# Autodesk Inventor assembly: Arm 2.0 Assembly
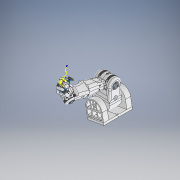
[picture p0: Inventor's stored thumbnail of the model, 180x180]
Saved by Autodesk Inventor 2017 SP1 (Build 210196100, 196)
## iProperties
Created: 2017-09-28
Part Number: Arm 2.0 Assembly
Document SubType Name: Assembly
Designer: Zach
Author: Zach
## Documents named in this file (39)
- C:\Users\Zach\Documents\GitHub\tr1\src\Body\Arm 2.0 Assembly\Arm 2.0 Assembly.iam
- C:\Users\Zach\Documents\GitHub\tr1\src\Body\Arm 2.0 Assembly\AA001.ipt
- C:\Users\Zach\Documents\GitHub\tr1\src\Body\Arm 2.0 Assembly\Steel Rod 8mm x 135mm.ipt
- C:\Users\Zach\Documents\GitHub\tr1\lib\22x8x8mm Bearing.ipt
- C:\Users\Zach\Documents\GitHub\tr1\src\Body\Arm 2.0 Assembly\AA002.ipt
- C:\Users\Zach\Documents\GitHub\tr1\src\Body\Arm 2.0 Assembly\AA003.ipt
- C:\Users\Zach\Documents\GitHub\tr1\src\Body\Arm 2.0 Assembly\AA004.ipt
- C:\Users\Zach\Documents\GitHub\tr1\src\Body\Arm 2.0 Assembly\AA005.ipt
- C:\Users\Zach\Documents\GitHub\tr1\src\Body\Arm 2.0 Assembly\AA006.ipt
- C:\Users\Zach\Documents\GitHub\tr1\src\Body\Arm 2.0 Assembly\AA007.ipt
- C:\Users\Zach\Documents\GitHub\tr1\lib\QS12MM250\QS12MM250.ipt
- C:\Users\Zach\Documents\GitHub\tr1\src\Body\Arm 2.0 Assembly\AA008.ipt
- C:\Users\Zach\Documents\GitHub\tr1\src\Body\Arm 2.0 Assembly\AA009.ipt
- C:\Users\Zach\Documents\GitHub\tr1\lib\13x4x5mm Bearing.ipt
- C:\Users\Zach\Documents\GitHub\tr1\src\Body\Arm 2.0 Assembly\AA010.ipt
- C:\Users\Zach\Documents\GitHub\tr1\src\Body\Arm 2.0 Assembly\AA011.ipt
- C:\Users\Zach\Documents\GitHub\tr1\src\Body\Arm 2.0 Assembly\AA012.ipt
- C:\Users\Zach\Documents\GitHub\tr1\src\Body\Arm 2.0 Assembly\Steel Rod 8mm x 100mm.ipt
- C:\Users\Zach\Documents\GitHub\tr1\src\Body\Arm 2.0 Assembly\AA013.ipt
- C:\Users\Zach\Documents\GitHub\tr1\src\Body\Arm 2.0 Assembly\AA014.ipt
- C:\Users\Zach\Documents\GitHub\tr1\src\Body\Arm 2.0 Assembly\AA015.ipt
- C:\Users\Zach\Documents\GitHub\tr1\src\Body\Arm 2.0 Assembly\AA016.ipt
- C:\Users\Zach\Documents\GitHub\tr1\src\Body\Arm 2.0 Assembly\AA017.ipt
- C:\Users\Zach\Documents\Inventor\Content Center Files\R2017\en-US\ISO 4762(2)\ISO 4762 - M4 x 20ISO.ipt
- C:\Users\Zach\Documents\Inventor\Content Center Files\R2017\en-US\ISO 4035(2)\ISO 4035 - M4 - ISO.ipt
- C:\Users\Zach\Documents\GitHub\tr1\lib\12V DC Motor 378-1.ipt
- C:\Users\Zach\Documents\GitHub\tr1\src\Body\Arm 2.0 Assembly\AA018.ipt
- C:\Users\Zach\Documents\Inventor\Content Center Files\R2017\en-US\ISO 4016\ISO 4016 - M5 x 25.ipt
- C:\Users\Zach\Documents\Inventor\Content Center Files\R2017\en-US\ISO 4017(1)\ISO 4017 - M5 x 12 - ISO.ipt
- C:\Users\Zach\Documents\Inventor\Content Center Files\R2017\en-US\ISO 4017(1)\ISO 4017 - M5 x 20 - ISO.ipt
- C:\Users\Zach\Documents\GitHub\tr1\src\Body\Arm 2.0 Assembly\AA019.ipt
- C:\Users\Zach\Documents\GitHub\tr1\src\Body\Arm 2.0 Assembly\AA020.ipt
- C:\Users\Zach\Documents\GitHub\tr1\src\Body\Arm 2.0 Assembly\AA021.ipt
- C:\Users\Zach\Documents\GitHub\tr1\src\Body\Arm 2.0 Assembly\AA022.ipt
- C:\Users\Zach\Documents\GitHub\tr1\src\Body\Arm 2.0 Assembly\Steel Rod 8mm x 80mm.ipt
- C:\Users\Zach\Documents\GitHub\tr1\src\Body\Arm 2.0 Assembly\AA023.ipt
- C:\Users\Zach\Documents\GitHub\BCN3D-Moveo\Autodesk Inventor files\Gripper B Assembly.iam
- C:\Users\Zach\Documents\GitHub\tr1\src\Body\Arm 2.0 Assembly\AA024.ipt
- C:\Users\Zach\Documents\GitHub\tr1\lib\Gearbox 8;1\Gearbox 8;1.iam
## Components (88 placed, 38 different names)
1. AA001:1 — Mate:1, Mate:3, Flush:1, Flush:2, Mate:7, Mate:9, Mate:10, Mate:11, Mate:58, Mate:59, Mate:60, Mate:61, Mate:62, Mate:63, Mate:82, Mate:83, Mate:84, Mate:101, Mate:102, Mate:104, Mate:105, Mate:138, Mate:139, Mate:140, Mate:141
2. AA002:2 — Flush:4, Mate:5, Mate:8, Mate:14, Mate:28, Mate:29, Mate:34
3. AA003:1 — Flush:4, Mate:5, Mate:6, Mate:7, Mate:8, Mate:27, Mate:32
4. AA004:1 — Mate:9, Mate:10, Mate:11, Mate:12, Mate:13, Mate:15, Mate:23, Mate:26
5. AA005:1 — Mate:26, Mate:99, Mate:100, Mate:103
6. AA006:1 — Mate:24, Mate:25, Mate:96, Mate:97, Mate:98
7. AA007:1 — Mate:19, Mate:20, Mate:99, Mate:100, Mate:103
8. AA007:2 — Mate:19, Mate:20, Mate:96, Mate:97, Mate:98
9. AA008:1 — Mate:27, Mate:28, Mate:29, Mate:30, Mate:31, Mate:33, Mate:35, Mate:36, Mate:39, Mate:41, Mate:43, Mate:46, Mate:47, Mate:131, Mate:132, Mate:135, Mate:137, Flush:11, Mate:167, Mate:213
10. AA008:2 — Mate:32, Mate:33, Mate:34, Mate:37, Mate:38, Mate:40, Mate:42, Mate:44, Mate:45, Mate:48, Mate:76, Mate:130, Mate:133, Mate:134, Mate:136, Flush:12, Mate:168, Mate:212, Mate:218, Mate:219, Mate:220
11. AA009:1 — Mate:30, Mate:31
12. AA010:1 — Mate:47, Mate:48, Mate:52, Mate:53, Mate:55, Flush:6, Mate:56, Flush:7, Flush:8, Mate:64, Mate:65, Mate:66, Mate:67, Mate:68, Mate:69, Mate:107, Mate:108, Mate:109, Mate:214
13. AA011:1 — Mate:49, Mate:50, Mate:51, Flush:9, Mate:79, Mate:81, Mate:113, Mate:114
14. AA012:1 — Mate:49, Mate:50, Mate:51, Mate:52, Mate:53, Flush:9, Mate:80, Mate:110, Mate:112, Mate:115
15. AA013:1 — Mate:58, Mate:59, Mate:60, Mate:148, Mate:149, Mate:150, Mate:151, Mate:152, Mate:153
16. AA013:2 — Mate:61, Mate:62, Mate:63, Mate:142, Mate:143, Mate:144, Mate:145, Mate:146, Mate:147
17. AA014:1 — Mate:64, Mate:65, Mate:66, Mate:160, Mate:161, Mate:162, Mate:163, Mate:164, Mate:165
18. AA014:2 — Mate:67, Mate:68, Mate:69, Mate:154, Mate:155, Mate:156, Mate:157, Mate:158, Mate:159
19. AA015:1 — Mate:166, Flush:11, Mate:167
20. AA015:2 — Mate:76, Flush:12, Mate:168
21. AA016:1 — Mate:79, Mate:80, Mate:81, Flush:10, Mate:111, Mate:112, Mate:113, Mate:116, Mate:124, Mate:125, Mate:127, Mate:129, Flush:14, Mate:170, Mate:215, Mate:216, Mate:217
22. AA016:2 — Flush:10, Mate:110, Mate:111, Mate:114, Mate:115, Mate:119, Mate:122, Mate:123, Mate:126, Mate:128, Flush:13, Mate:169, Mate:180, Mate:181
23. AA017:1 — Mate:82, Mate:83, Mate:84, Mate:85, Mate:86, Mate:91, Mate:92, Mate:95
24. AA018:1 — Mate:116, Flush:14, Mate:170
25. AA018:2 — Mate:119, Flush:13, Mate:169
26. AA019:1 — Mate:174, Mate:175, Mate:176, Mate:177, Mate:178, Mate:179, Mate:182, Mate:183, Mate:184, Mate:185, Flush:15, Flush:16, Flush:17, Mate:188, Mate:189, Mate:190, Mate:191, Mate:192, Mate:193
27. AA020:1 — Mate:171, Mate:172, Mate:173, Mate:175, Mate:194, Mate:196
28. AA021:1 — Mate:171, Mate:172, Mate:173, Mate:174, Mate:195
29. AA022:1 — Mate:176, Mate:177, Mate:181, Mate:200, Flush:18, Mate:203, Mate:204, Mate:206, Mate:209, Mate:210
30. AA022:2 — Mate:178, Mate:179, Mate:180, Flush:19, Mate:201, Mate:202, Mate:205, Mate:207, Mate:208, Mate:211
31. AA023:1 — Mate:188, Mate:189, Mate:193
32. AA023:2 — Mate:190, Mate:191, Mate:192
33. AA024:1 — Mate:200, Flush:18, Mate:203
34. AA024:2 — Flush:19, Mate:201, Mate:202
35. Gearbox 8;1:1 [sub-assembly] — Mate:212, Mate:213, Mate:214
36. Gripper B Assembly:1 [sub-assembly] — Mate:194, Mate:195, Mate:196
37. 13x4x5mm Bearing:1 — Mate:35, Mate:36
38. 13x4x5mm Bearing:2 — Mate:37, Mate:38
39. 13x4x5mm Bearing:3 — Mate:40, Mate:44
40. 13x4x5mm Bearing:4 — Mate:39, Mate:43
41. 13x4x5mm Bearing:5 — Mate:42, Mate:45
42. 13x4x5mm Bearing:6 — Mate:41, Mate:46
43. 13x4x5mm Bearing:7 — Mate:85, Mate:86, Mate:87, Mate:88, Mate:94
44. 13x4x5mm Bearing:8 — Mate:89, Mate:90
45. 13x4x5mm Bearing:9 — Mate:87, Mate:88, Mate:89, Mate:90
46. 22x8x8mm Bearing:1 — Mate:3, Flush:1, Flush:3
47. 22x8x8mm Bearing:2 — Flush:2, Mate:105
48. 22x8x8mm Bearing:3 — Mate:55, Flush:6, Mate:57
49. 22x8x8mm Bearing:4 — Mate:56, Flush:7
50. 22x8x8mm Bearing:5 — Mate:186, Flush:16
51. 22x8x8mm Bearing:6 — Mate:187, Flush:17
52. QS12MM250:1 — Mate:23, Mate:24, Mate:25
53. Steel Rod 8mm x 135mm:1 — Mate:1, Flush:3, Mate:6
54. Steel Rod 8mm x 100mm:1 — Mate:57, Flush:8
55. Steel Rod 8mm x 80mm:1 — Mate:185, Flush:15, Mate:186, Mate:187
56. 12V DC Motor 378-1:1 — Mate:101, Mate:102, Mate:104
57. 12V DC Motor 378-1:2 — Mate:107, Mate:108, Mate:109
58. 12V DC Motor 378-1:3 — Mate:182, Mate:183, Mate:184
59. 12V DC Motor 378-1:4 — Mate:215, Mate:216, Mate:217
60. 12V DC Motor 378-1:5 — Mate:218, Mate:219, Mate:220
61. ISO 4762 M4 x 20:1 — Mate:91, Mate:92, Mate:93
62. ISO 4035 M4:1 — Mate:93, Mate:94, Mate:95
63. ISO 4016 M5 x 25:1 — Mate:122, Mate:123
64. ISO 4016 M5 x 25:2 — Mate:124, Mate:125
65. ISO 4016 M5 x 25:3 — Mate:127, Mate:129
66. ISO 4016 M5 x 25:4 — Mate:126, Mate:128
67. ISO 4016 M5 x 25:5 — Mate:130, Mate:133
68. ISO 4016 M5 x 25:6 — Mate:131, Mate:132
69. ISO 4016 M5 x 25:7 — Mate:134, Mate:136
70. ISO 4016 M5 x 25:8 — Mate:135, Mate:137, Mate:166
71. ISO 4016 M5 x 25:9 — Mate:138, Mate:139
72. ISO 4016 M5 x 25:10 — Mate:140, Mate:141
73. ISO 4016 M5 x 25:11 — Mate:204, Mate:206
74. ISO 4016 M5 x 25:12 — Mate:205, Mate:207
75. ISO 4017 M5 x 20:1 — Mate:146, Mate:147
76. ISO 4017 M5 x 20:2 — Mate:144, Mate:145
77. ISO 4017 M5 x 20:3 — Mate:142, Mate:143
78. ISO 4017 M5 x 20:4 — Mate:148, Mate:149
79. ISO 4017 M5 x 20:5 — Mate:152, Mate:153
80. ISO 4017 M5 x 20:6 — Mate:150, Mate:151
81. ISO 4017 M5 x 12:1 — Mate:154, Mate:155
82. ISO 4017 M5 x 12:2 — Mate:156, Mate:158
83. ISO 4017 M5 x 12:3 — Mate:157, Mate:159
84. ISO 4017 M5 x 12:4 — Mate:160, Mate:161
85. ISO 4017 M5 x 12:5 — Mate:162, Mate:163
86. ISO 4017 M5 x 12:6 — Mate:164, Mate:165
87. ISO 4016 M5 x 25:13 — Mate:209, Mate:210
88. ISO 4016 M5 x 25:14 — Mate:208, Mate:211
## Relationships (214: Mate 196, Flush 18)
- Mate:1: AA001:1 ↔ Steel Rod 8mm x 135mm:1
- Mate:3: AA001:1 ↔ 22x8x8mm Bearing:1
- Flush:1: AA001:1 ↔ 22x8x8mm Bearing:1
- Flush:2: AA001:1 ↔ 22x8x8mm Bearing:2
- Flush:3 (-2.5 mm): 22x8x8mm Bearing:1 ↔ Steel Rod 8mm x 135mm:1
- Flush:4: AA002:2 ↔ AA003:1
- Mate:5: AA002:2 ↔ AA003:1
- Mate:6: AA003:1 ↔ Steel Rod 8mm x 135mm:1
- Mate:7 (0.75 mm): AA001:1 ↔ AA003:1
- Mate:8: AA002:2 ↔ AA003:1
- Mate:9: AA001:1 ↔ AA004:1
- Mate:10: AA001:1 ↔ AA004:1
- Mate:11: AA001:1 ↔ AA004:1
- Mate:12: AA004:1
- Mate:13: AA004:1
- Mate:14: AA002:2
- Mate:15: AA004:1
- Mate:19: AA007:1 ↔ AA007:2
- Mate:20: AA007:1 ↔ AA007:2
- Mate:23: AA004:1 ↔ QS12MM250:1
- Mate:24: AA006:1 ↔ QS12MM250:1
- Mate:25: AA006:1 ↔ QS12MM250:1
- Mate:26 (30 mm): AA004:1 ↔ AA005:1
- Mate:27: AA003:1 ↔ AA008:1
- Mate:28: AA002:2 ↔ AA008:1
- Mate:29: AA002:2 ↔ AA008:1
- Mate:30: AA008:1 ↔ AA009:1
- Mate:31: AA008:1 ↔ AA009:1
- Mate:32: AA003:1 ↔ AA008:2
- Mate:33: AA008:1 ↔ AA008:2
- Mate:34: AA002:2 ↔ AA008:2
- Mate:35: AA008:1 ↔ 13x4x5mm Bearing:1
- Mate:36: AA008:1 ↔ 13x4x5mm Bearing:1
- Mate:37: AA008:2 ↔ 13x4x5mm Bearing:2
- Mate:38: AA008:2 ↔ 13x4x5mm Bearing:2
- Mate:39: AA008:1 ↔ 13x4x5mm Bearing:4
- Mate:40: AA008:2 ↔ 13x4x5mm Bearing:3
- Mate:41: AA008:1 ↔ 13x4x5mm Bearing:6
- Mate:42: AA008:2 ↔ 13x4x5mm Bearing:5
- Mate:43: AA008:1 ↔ 13x4x5mm Bearing:4
- Mate:44: AA008:2 ↔ 13x4x5mm Bearing:3
- Mate:45: AA008:2 ↔ 13x4x5mm Bearing:5
- Mate:46: AA008:1 ↔ 13x4x5mm Bearing:6
- Mate:47: AA008:1 ↔ AA010:1
- Mate:48 (2.5 mm): AA008:2 ↔ AA010:1
- Mate:49: AA011:1 ↔ AA012:1
- Mate:50: AA011:1 ↔ AA012:1
- Mate:51: AA011:1 ↔ AA012:1
- Mate:52: AA010:1 ↔ AA012:1
- Mate:53 (1.75 mm): AA010:1 ↔ AA012:1
- Mate:55: AA010:1 ↔ 22x8x8mm Bearing:3
- Flush:6: AA010:1 ↔ 22x8x8mm Bearing:3
- Mate:56: AA010:1 ↔ 22x8x8mm Bearing:4
- Flush:7: AA010:1 ↔ 22x8x8mm Bearing:4
- Mate:57: 22x8x8mm Bearing:3 ↔ Steel Rod 8mm x 100mm:1
- Flush:8 (2.5 mm): AA010:1 ↔ Steel Rod 8mm x 100mm:1
- Mate:58: AA001:1 ↔ AA013:1
- Mate:59: AA001:1 ↔ AA013:1
- Mate:60: AA001:1 ↔ AA013:1
- Mate:61: AA001:1 ↔ AA013:2
- Mate:62: AA001:1 ↔ AA013:2
- Mate:63: AA001:1 ↔ AA013:2
- Mate:64: AA010:1 ↔ AA014:1
- Mate:65: AA010:1 ↔ AA014:1
- Mate:66: AA010:1 ↔ AA014:1
- Mate:67: AA010:1 ↔ AA014:2
- Mate:68: AA010:1 ↔ AA014:2
- Mate:69: AA010:1 ↔ AA014:2
- Mate:76: AA008:2 ↔ AA015:2
- Flush:9: AA011:1 ↔ AA012:1
- Mate:79: AA011:1 ↔ AA016:1
- Mate:80: AA012:1 ↔ AA016:1
- Mate:81: AA011:1 ↔ AA016:1
- Mate:82: AA001:1 ↔ AA017:1
- Mate:83: AA001:1 ↔ AA017:1
- Mate:84: AA001:1 ↔ AA017:1
- Mate:85: AA017:1 ↔ 13x4x5mm Bearing:7
- Mate:86 (0.5 mm): AA017:1 ↔ 13x4x5mm Bearing:7
- Mate:87: 13x4x5mm Bearing:7 ↔ 13x4x5mm Bearing:9
- Mate:88: 13x4x5mm Bearing:7 ↔ 13x4x5mm Bearing:9
- Mate:89: 13x4x5mm Bearing:8 ↔ 13x4x5mm Bearing:9
- Mate:90: 13x4x5mm Bearing:8 ↔ 13x4x5mm Bearing:9
- Mate:91: AA017:1 ↔ ISO 4762 M4 x 20:1
- Mate:92: AA017:1 ↔ ISO 4762 M4 x 20:1
- Mate:93: ISO 4762 M4 x 20:1 ↔ ISO 4035 M4:1
- Mate:94: 13x4x5mm Bearing:7 ↔ ISO 4035 M4:1
- Mate:95: AA017:1 ↔ ISO 4035 M4:1
- Mate:96: AA006:1 ↔ AA007:2
- Mate:97: AA006:1 ↔ AA007:2
- Mate:98: AA006:1 ↔ AA007:2
- Mate:99: AA005:1 ↔ AA007:1
- Mate:100: AA005:1 ↔ AA007:1
- Mate:101: AA001:1 ↔ 12V DC Motor 378-1:1
- Mate:102: AA001:1 ↔ 12V DC Motor 378-1:1
- Mate:103: AA005:1 ↔ AA007:1
- Mate:104: AA001:1 ↔ 12V DC Motor 378-1:1
- Mate:105: AA001:1 ↔ 22x8x8mm Bearing:2
- Mate:107: AA010:1 ↔ 12V DC Motor 378-1:2
- Mate:108: AA010:1 ↔ 12V DC Motor 378-1:2
- Mate:109: AA010:1 ↔ 12V DC Motor 378-1:2
- Flush:10: AA016:1 ↔ AA016:2
- Mate:110: AA012:1 ↔ AA016:2
- Mate:111: AA016:1 ↔ AA016:2
- Mate:112: AA012:1 ↔ AA016:1
- Mate:113: AA011:1 ↔ AA016:1
- Mate:114: AA011:1 ↔ AA016:2
- Mate:115: AA012:1 ↔ AA016:2
- Mate:116: AA016:1 ↔ AA018:1
- Mate:119: AA016:2 ↔ AA018:2
- Mate:122: AA016:2 ↔ ISO 4016 M5 x 25:1
- Mate:123: AA016:2 ↔ ISO 4016 M5 x 25:1
- Mate:124: AA016:1 ↔ ISO 4016 M5 x 25:2
- Mate:125: AA016:1 ↔ ISO 4016 M5 x 25:2
- Mate:126: AA016:2 ↔ ISO 4016 M5 x 25:4
- Mate:127: AA016:1 ↔ ISO 4016 M5 x 25:3
- Mate:128: AA016:2 ↔ ISO 4016 M5 x 25:4
- Mate:129: AA016:1 ↔ ISO 4016 M5 x 25:3
- Mate:130: AA008:2 ↔ ISO 4016 M5 x 25:5
- Mate:131: AA008:1 ↔ ISO 4016 M5 x 25:6
- Mate:132: AA008:1 ↔ ISO 4016 M5 x 25:6
- Mate:133: AA008:2 ↔ ISO 4016 M5 x 25:5
- Mate:134: AA008:2 ↔ ISO 4016 M5 x 25:7
- Mate:135: AA008:1 ↔ ISO 4016 M5 x 25:8
- Mate:136: AA008:2 ↔ ISO 4016 M5 x 25:7
- Mate:137: AA008:1 ↔ ISO 4016 M5 x 25:8
- Mate:138: AA001:1 ↔ ISO 4016 M5 x 25:9
- Mate:139: AA001:1 ↔ ISO 4016 M5 x 25:9
- Mate:140: AA001:1 ↔ ISO 4016 M5 x 25:10
- Mate:141: AA001:1 ↔ ISO 4016 M5 x 25:10
- Mate:142: AA013:2 ↔ ISO 4017 M5 x 20:3
- Mate:143: AA013:2 ↔ ISO 4017 M5 x 20:3
- Mate:144: AA013:2 ↔ ISO 4017 M5 x 20:2
- Mate:145: AA013:2 ↔ ISO 4017 M5 x 20:2
- Mate:146: AA013:2 ↔ ISO 4017 M5 x 20:1
- Mate:147: AA013:2 ↔ ISO 4017 M5 x 20:1
- Mate:148: AA013:1 ↔ ISO 4017 M5 x 20:4
- Mate:149: AA013:1 ↔ ISO 4017 M5 x 20:4
- Mate:150: AA013:1 ↔ ISO 4017 M5 x 20:6
- Mate:151: AA013:1 ↔ ISO 4017 M5 x 20:6
- Mate:152: AA013:1 ↔ ISO 4017 M5 x 20:5
- Mate:153: AA013:1 ↔ ISO 4017 M5 x 20:5
- Mate:154: AA014:2 ↔ ISO 4017 M5 x 12:1
- Mate:155: AA014:2 ↔ ISO 4017 M5 x 12:1
- Mate:156: AA014:2 ↔ ISO 4017 M5 x 12:2
- Mate:157: AA014:2 ↔ ISO 4017 M5 x 12:3
- Mate:158: AA014:2 ↔ ISO 4017 M5 x 12:2
- Mate:159: AA014:2 ↔ ISO 4017 M5 x 12:3
- Mate:160: AA014:1 ↔ ISO 4017 M5 x 12:4
- Mate:161: AA014:1 ↔ ISO 4017 M5 x 12:4
- Mate:162: AA014:1 ↔ ISO 4017 M5 x 12:5
- Mate:163: AA014:1 ↔ ISO 4017 M5 x 12:5
- Mate:164: AA014:1 ↔ ISO 4017 M5 x 12:6
- Mate:165: AA014:1 ↔ ISO 4017 M5 x 12:6
- Mate:166: AA015:1 ↔ ISO 4016 M5 x 25:8
- Flush:11: AA008:1 ↔ AA015:1
- Mate:167 (1 mm): AA008:1 ↔ AA015:1
- Flush:12: AA008:2 ↔ AA015:2
- Mate:168 (1 mm): AA008:2 ↔ AA015:2
- Flush:13: AA016:2 ↔ AA018:2
- Mate:169 (1 mm): AA016:2 ↔ AA018:2
- Flush:14: AA016:1 ↔ AA018:1
- Mate:170 (1 mm): AA016:1 ↔ AA018:1
- Mate:171: AA020:1 ↔ AA021:1
- Mate:172: AA020:1 ↔ AA021:1
- Mate:173: AA020:1 ↔ AA021:1
- Mate:174 (1 mm): AA019:1 ↔ AA021:1
- Mate:175: AA019:1 ↔ AA020:1
- Mate:176: AA019:1 ↔ AA022:1
- Mate:177: AA019:1 ↔ AA022:1
- Mate:178: AA019:1 ↔ AA022:2
- Mate:179: AA019:1 ↔ AA022:2
- Mate:180: AA016:2 ↔ AA022:2
- Mate:181 (2.5 mm): AA016:2 ↔ AA022:1
- Mate:182: AA019:1 ↔ 12V DC Motor 378-1:3
- Mate:183: AA019:1 ↔ 12V DC Motor 378-1:3
- Mate:184: AA019:1 ↔ 12V DC Motor 378-1:3
- Mate:185: AA019:1 ↔ Steel Rod 8mm x 80mm:1
- Flush:15: AA019:1 ↔ Steel Rod 8mm x 80mm:1
- Mate:186: 22x8x8mm Bearing:5 ↔ Steel Rod 8mm x 80mm:1
- Flush:16: AA019:1 ↔ 22x8x8mm Bearing:5
- Mate:187: 22x8x8mm Bearing:6 ↔ Steel Rod 8mm x 80mm:1
- Flush:17: AA019:1 ↔ 22x8x8mm Bearing:6
- Mate:188: AA019:1 ↔ AA023:1
- Mate:189: AA019:1 ↔ AA023:1
- Mate:190: AA019:1 ↔ AA023:2
- Mate:191: AA019:1 ↔ AA023:2
- Mate:192: AA019:1 ↔ AA023:2
- Mate:193: AA019:1 ↔ AA023:1
- Mate:194: AA020:1 ↔ Gripper B Assembly:1
- Mate:195: AA021:1 ↔ Gripper B Assembly:1
- Mate:196: AA020:1 ↔ Gripper B Assembly:1
- Mate:200: AA022:1 ↔ AA024:1
- Flush:18: AA022:1 ↔ AA024:1
- Flush:19: AA022:2 ↔ AA024:2
- Mate:201: AA022:2 ↔ AA024:2
- Mate:202 (1 mm): AA022:2 ↔ AA024:2
- Mate:203 (1 mm): AA022:1 ↔ AA024:1
- Mate:204: AA022:1 ↔ ISO 4016 M5 x 25:11
- Mate:205: AA022:2 ↔ ISO 4016 M5 x 25:12
- Mate:206: AA022:1 ↔ ISO 4016 M5 x 25:11
- Mate:207: AA022:2 ↔ ISO 4016 M5 x 25:12
- Mate:208: AA022:2 ↔ ISO 4016 M5 x 25:14
- Mate:209: AA022:1 ↔ ISO 4016 M5 x 25:13
- Mate:210: AA022:1 ↔ ISO 4016 M5 x 25:13
- Mate:211: AA022:2 ↔ ISO 4016 M5 x 25:14
- Mate:212: AA008:2 ↔ Gearbox 8;1:1
- Mate:213: AA008:1 ↔ Gearbox 8;1:1
- Mate:214: AA010:1 ↔ Gearbox 8;1:1
- Mate:215: AA016:1 ↔ 12V DC Motor 378-1:4
- Mate:216: AA016:1 ↔ 12V DC Motor 378-1:4
- Mate:217: AA016:1 ↔ 12V DC Motor 378-1:4
- Mate:218: AA008:2 ↔ 12V DC Motor 378-1:5
- Mate:219: AA008:2 ↔ 12V DC Motor 378-1:5
- Mate:220: AA008:2 ↔ 12V DC Motor 378-1:5
